# Autodesk Inventor assembly: capacitor
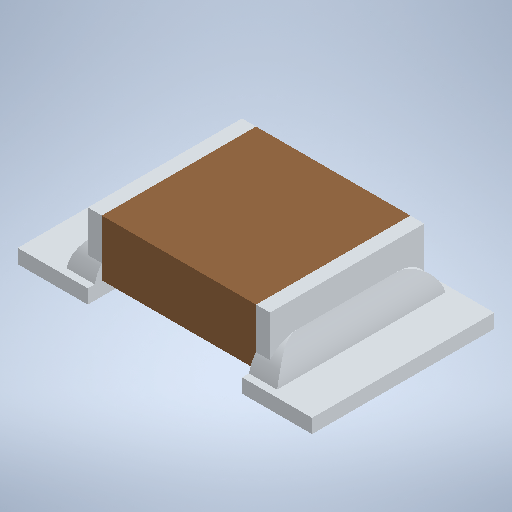
[picture p0: Inventor's stored thumbnail of the model, 512x512]
Saved by Autodesk Inventor 2025 (Build 290162000, 162)
## iProperties
Created: 2025-09-09
Part Number: capacitor
Document SubType Name: Assembly
Designer: jirne
Author: jirne
## Documents named in this file (3)
- C:\Users\jirne\JVR11\hardware\library\3D\DCJ11\capacitor\capacitor.iam
- C:\Users\jirne\JVR11\hardware\library\3D\DCJ11\capacitor\body.ipt
- C:\Users\jirne\JVR11\hardware\library\3D\DCJ11\capacitor\connection.ipt
## Components (3 placed, 2 different names)
1. body:1 — Mate:1, Mate:2, Mate:3, Mate:4
2. connection:1 — Mate:1, Mate:2
3. connection:2 — Mate:3, Mate:4
## Relationships (4: Mate 4)
- Mate:1: body:1 ↔ connection:1
- Mate:2: body:1 ↔ connection:1
- Mate:3: body:1 ↔ connection:2
- Mate:4: body:1 ↔ connection:2
